# Autodesk Inventor assembly: printer2
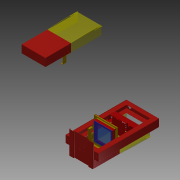
[picture p0: Inventor's stored thumbnail of the model, 180x180]
Saved by Autodesk Inventor 2014 SP2 (Build 180246200, 246)
## iProperties
Created: 2016-06-19
Part Number: printer2
Document SubType Name: Assembly
Designer: cruiser
Author: cruiser
## Documents named in this file (12)
- C:\Users\cruiser\Desktop\models\3d printers\laserresin4\printer2.iam
- C:\Users\cruiser\Desktop\models\3d printers\laserresin4\carrier2.ipt
- C:\Users\cruiser\Desktop\models\3d printers\laserresin4\frame_face2.ipt
- C:\Users\cruiser\Desktop\models\3d printers\laserresin4\door_assembly.iam
- C:\Users\cruiser\Desktop\models\3d printers\laserresin4\shf8.ipt
- C:\Users\cruiser\Desktop\models\3d printers\laserresin4\frame_back.ipt
- C:\Users\cruiser\Desktop\models\3d printers\laserresin4\crane_assembly.iam
- C:\Users\cruiser\Desktop\models\3d printers\laserresin4\reservoir.ipt
- C:\Users\cruiser\Desktop\models\3d printers\laserresin4\tray.ipt
- C:\Users\cruiser\Desktop\models\3d printers\laserresin4\laserholder.ipt
- C:\Users\cruiser\Desktop\models\3d printers\laserresin4\frame_feet.ipt
- C:\Users\cruiser\Desktop\models\3d printers\laserresin4\subframe.ipt
## Components (13 placed, 11 different names)
1. carrier2:1 — Mate:3, Mate:4, Mate:14, Mate:15, Mate:16
2. frame_face2:1 — Mate:1, Mate:2, Mate:5, Mate:6, Mate:7, Mate:8, Mate:9, Mate:10, Mate:11, Mate:12, Mate:13
3. door_assembly:1 [sub-assembly]
4. shf8:1 — Mate:1, Mate:2
5. frame_back:1
6. crane_assembly:1 [sub-assembly]
7. reservoir:1 — Mate:14, Mate:15, Mate:16, Mate:17, Mate:18, Mate:19
8. tray:1 — Mate:17, Mate:18, Mate:19
9. shf8:2 — Mate:3, Mate:4
10. laserholder:1 — Mate:11, Mate:12, Mate:13
11. frame_feet:1 — Mate:5, Mate:6, Mate:7
12. subframe:1 — Mate:8, Mate:9, Mate:10
13. door_assembly:2 [sub-assembly]
## Relationships (19: Mate 19)
- Mate:1: frame_face2:1 ↔ shf8:1
- Mate:2: frame_face2:1 ↔ shf8:1
- Mate:3: carrier2:1 ↔ shf8:2
- Mate:4: carrier2:1 ↔ shf8:2
- Mate:5: frame_face2:1 ↔ frame_feet:1
- Mate:6: frame_face2:1 ↔ frame_feet:1
- Mate:7: frame_face2:1 ↔ frame_feet:1
- Mate:8: frame_face2:1 ↔ subframe:1
- Mate:9: frame_face2:1 ↔ subframe:1
- Mate:10: frame_face2:1 ↔ subframe:1
- Mate:11: frame_face2:1 ↔ laserholder:1
- Mate:12: frame_face2:1 ↔ laserholder:1
- Mate:13: frame_face2:1 ↔ laserholder:1
- Mate:14: carrier2:1 ↔ reservoir:1
- Mate:15: carrier2:1 ↔ reservoir:1
- Mate:16: carrier2:1 ↔ reservoir:1
- Mate:17: reservoir:1 ↔ tray:1
- Mate:18: reservoir:1 ↔ tray:1
- Mate:19: reservoir:1 ↔ tray:1
